# Autodesk Inventor assembly: left_leg_MIR
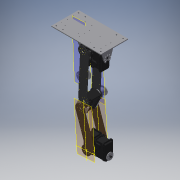
[picture p0: Inventor's stored thumbnail of the model, 180x180]
Saved by Autodesk Inventor 2018 (Build 220112000, 112)
## iProperties
Created: 2018-11-26
Part Number: left_leg_MIR
Document SubType Name: Assembly
Designer: bitbots
Mass: 578.906 g
Surface Area: 2185.74 cm^2
Volume: 578.906 cm^3
Density: 1 g/cm^3
Author: bitbots
## Documents named in this file (14)
- C:\Users\bitbots\Desktop\bitbots_hardware\wolfgang\assembly\legs\left_leg.iam
- C:\Users\bitbots\Desktop\bitbots_hardware\wolfgang\assembly\legs\lower_leg_MIR.ipt
- C:\Users\bitbots\Desktop\bitbots_hardware\wolfgang\assembly\legs\upper_leg_MIR.ipt
- C:\Users\bitbots\Desktop\bitbots_hardware\wolfgang\assembly\motors\MX106\MX-106_with_bearing_MIR.iam
- C:\Users\bitbots\Desktop\bitbots_hardware\wolfgang\assembly\legs\knee_connector_MIR.ipt
- C:\Users\bitbots\Desktop\bitbots_hardware\wolfgang\assembly\legs\motor_connector_MIR.ipt
- C:\Users\bitbots\Desktop\bitbots_hardware\wolfgang\assembly\motors\MX106\MX-106_with_horn_MIR.iam
- C:\Users\bitbots\Desktop\bitbots_hardware\wolfgang\assembly\legs\ankle_MIR.ipt
- C:\Users\bitbots\Desktop\bitbots_hardware\wolfgang\assembly\legs\foot_MIR.ipt
- C:\Users\bitbots\Documents\spring_holder.ipt
- C:\Users\bitbots\Documents\springerholder_top.ipt
- C:\Users\bitbots\Documents\spring_holder_lower.ipt
- C:\Users\bitbots\Documents\springholder_new.ipt
- C:\Users\bitbots\Documents\springholder_new_bottom.ipt
## Components (22 placed, 13 different names)
1. lower_leg_MIR:1 — Mate:41, Mate:40, Mate:39, Mate:58, Mate:57, Flush:1, Flush:2, Flush:3, Flush:4, Flush:5, Flush:6, Mate:71, Mate:72, Mate:73
2. upper_leg_MIR:1 — Mate:33, Mate:32, Mate:31, Mate:35, Mate:34
3. lower_leg_MIR:2 — Mate:81, Mate:61, Mate:80, Mate:64
4. upper_leg_MIR:2 — Mate:82, Mate:28, Mate:38, Mate:37, Mate:36, Mate:52
5. MX-106_with_bearing_MIR:1 [sub-assembly] — Mate:81, Mate:61, Mate:41, Mate:40, Mate:39, Mate:22, Mate:21, Mate:20, Mate:18, Mate:17, Mate:16
6. MX-106_with_bearing_MIR:2 [sub-assembly] — Mate:82, Mate:33, Mate:32, Mate:31, Mate:29, Mate:28, Mate:10, Mate:9, Mate:8, Mate:7, Mate:6, Mate:5
7. knee_connector_MIR:1 — Mate:38, Mate:37, Mate:36, Mate:22, Mate:21, Mate:20, Mate:52
8. knee_connector_MIR:2 — Mate:35, Mate:34, Mate:18, Mate:17, Mate:16
9. motor_connector_MIR:1 — Mate:54, Mate:55, Mate:56, Mate:59, Mate:60, Mate:64
10. motor_connector_MIR:2 — Mate:73, Mate:57, Mate:58, Mate:61, Mate:62, Mate:63
11. motor_connector_MIR:3 — Mate:10, Mate:9, Mate:8, Mate:12, Mate:11
12. motor_connector_MIR:4 — Mate:7, Mate:6, Mate:5, Mate:13
13. MX-106_with_horn_MIR:1 [sub-assembly] — Mate:30, Mate:13, Mate:12, Mate:11, Angle:2
14. MX-106_with_bearing_MIR:3 [sub-assembly] — Mate:80, Mate:64, Mate:58, Mate:57, Mate:59, Mate:60, Mate:64
15. MX-106_with_horn_MIR:2 [sub-assembly] — Mate:73, Mate:54, Mate:55, Mate:56, Mate:57, Mate:58, Mate:61, Mate:62, Mate:63, Mate:65, Mate:66, Mate:67, Angle:2
16. ankle_MIR:1 — Mate:79, Mate:78, Mate:77, Mate:65, Mate:66, Mate:67
17. foot_MIR:1 — Mate:79, Mate:78, Mate:77, Angle:1
18. spring_holder:1 — Flush:1, Flush:2, Mate:68, Mate:69, Mate:70
19. springerholder_top:1 — Mate:68, Mate:69, Mate:70
20. spring_holder_lower:1 — Flush:3, Flush:4
21. springholder_new:1 — Flush:5, Flush:6, Mate:74, Mate:75, Mate:76
22. springholder_new_bottom:1 — Mate:71, Mate:72, Mate:73, Mate:74, Mate:75, Mate:76
## Relationships (72: Mate 64, Flush 6, Angle 2)
- Mate:81: lower_leg_MIR:2 ↔ MX-106_with_bearing_MIR:1
- Mate:61: lower_leg_MIR:2 ↔ MX-106_with_bearing_MIR:1
- Mate:41: lower_leg_MIR:1 ↔ MX-106_with_bearing_MIR:1
- Mate:40: lower_leg_MIR:1 ↔ MX-106_with_bearing_MIR:1
- Mate:39: lower_leg_MIR:1 ↔ MX-106_with_bearing_MIR:1
- Mate:82: upper_leg_MIR:2 ↔ MX-106_with_bearing_MIR:2
- Mate:33: upper_leg_MIR:1 ↔ MX-106_with_bearing_MIR:2
- Mate:32: upper_leg_MIR:1 ↔ MX-106_with_bearing_MIR:2
- Mate:31: upper_leg_MIR:1 ↔ MX-106_with_bearing_MIR:2
- Mate:29: MX-106_with_bearing_MIR:2
- Mate:28: upper_leg_MIR:2 ↔ MX-106_with_bearing_MIR:2
- Mate:38 (0.65 mm): upper_leg_MIR:2 ↔ knee_connector_MIR:1
- Mate:37: upper_leg_MIR:2 ↔ knee_connector_MIR:1
- Mate:36: upper_leg_MIR:2 ↔ knee_connector_MIR:1
- Mate:22: MX-106_with_bearing_MIR:1 ↔ knee_connector_MIR:1
- Mate:21: MX-106_with_bearing_MIR:1 ↔ knee_connector_MIR:1
- Mate:20: MX-106_with_bearing_MIR:1 ↔ knee_connector_MIR:1
- Mate:35: upper_leg_MIR:1 ↔ knee_connector_MIR:2
- Mate:34: upper_leg_MIR:1 ↔ knee_connector_MIR:2
- Mate:18: MX-106_with_bearing_MIR:1 ↔ knee_connector_MIR:2
- Mate:17: MX-106_with_bearing_MIR:1 ↔ knee_connector_MIR:2
- Mate:16: MX-106_with_bearing_MIR:1 ↔ knee_connector_MIR:2
- Mate:10: MX-106_with_bearing_MIR:2 ↔ motor_connector_MIR:3
- Mate:9: MX-106_with_bearing_MIR:2 ↔ motor_connector_MIR:3
- Mate:8: MX-106_with_bearing_MIR:2 ↔ motor_connector_MIR:3
- Mate:7: MX-106_with_bearing_MIR:2 ↔ motor_connector_MIR:4
- Mate:6: MX-106_with_bearing_MIR:2 ↔ motor_connector_MIR:4
- Mate:5: MX-106_with_bearing_MIR:2 ↔ motor_connector_MIR:4
- Mate:30: MX-106_with_horn_MIR:1
- Mate:13: motor_connector_MIR:4 ↔ MX-106_with_horn_MIR:1
- Mate:12: motor_connector_MIR:3 ↔ MX-106_with_horn_MIR:1
- Mate:11: motor_connector_MIR:3 ↔ MX-106_with_horn_MIR:1
- Mate:80: lower_leg_MIR:2 ↔ MX-106_with_bearing_MIR:3
- Mate:64: lower_leg_MIR:2 ↔ MX-106_with_bearing_MIR:3
- Mate:58: lower_leg_MIR:1 ↔ MX-106_with_bearing_MIR:3
- Mate:57: lower_leg_MIR:1 ↔ MX-106_with_bearing_MIR:3
- Mate:73: motor_connector_MIR:2 ↔ MX-106_with_horn_MIR:2
- Mate:79: ankle_MIR:1 ↔ foot_MIR:1
- Mate:78: ankle_MIR:1 ↔ foot_MIR:1
- Mate:77: ankle_MIR:1 ↔ foot_MIR:1
- Mate:52 (0.65 mm): upper_leg_MIR:2 ↔ knee_connector_MIR:1
- Mate:54: motor_connector_MIR:1 ↔ MX-106_with_horn_MIR:2
- Mate:55: motor_connector_MIR:1 ↔ MX-106_with_horn_MIR:2
- Mate:56: motor_connector_MIR:1 ↔ MX-106_with_horn_MIR:2
- Mate:57: motor_connector_MIR:2 ↔ MX-106_with_horn_MIR:2
- Mate:58: motor_connector_MIR:2 ↔ MX-106_with_horn_MIR:2
- Mate:59: motor_connector_MIR:1 ↔ MX-106_with_bearing_MIR:3
- Mate:60: motor_connector_MIR:1 ↔ MX-106_with_bearing_MIR:3
- Mate:61: motor_connector_MIR:2 ↔ MX-106_with_horn_MIR:2
- Mate:62: motor_connector_MIR:2 ↔ MX-106_with_horn_MIR:2
- Mate:63: motor_connector_MIR:2 ↔ MX-106_with_horn_MIR:2
- Mate:64: motor_connector_MIR:1 ↔ MX-106_with_bearing_MIR:3
- Angle:1 (0 deg): foot_MIR:1
- Mate:65: MX-106_with_horn_MIR:2 ↔ ankle_MIR:1
- Mate:66: MX-106_with_horn_MIR:2 ↔ ankle_MIR:1
- Mate:67: MX-106_with_horn_MIR:2 ↔ ankle_MIR:1
- Flush:1: lower_leg_MIR:1 ↔ spring_holder:1
- Flush:2: lower_leg_MIR:1 ↔ spring_holder:1
- Mate:68: spring_holder:1 ↔ springerholder_top:1
- Mate:69: spring_holder:1 ↔ springerholder_top:1
- Mate:70: spring_holder:1 ↔ springerholder_top:1
- Flush:3: lower_leg_MIR:1 ↔ spring_holder_lower:1
- Flush:4: lower_leg_MIR:1 ↔ spring_holder_lower:1
- Angle:2 (0 deg): MX-106_with_horn_MIR:1 ↔ MX-106_with_horn_MIR:2
- Flush:5: lower_leg_MIR:1 ↔ springholder_new:1
- Flush:6: lower_leg_MIR:1 ↔ springholder_new:1
- Mate:71: lower_leg_MIR:1 ↔ springholder_new_bottom:1
- Mate:72: lower_leg_MIR:1 ↔ springholder_new_bottom:1
- Mate:73: lower_leg_MIR:1 ↔ springholder_new_bottom:1
- Mate:74: springholder_new:1 ↔ springholder_new_bottom:1
- Mate:75: springholder_new:1 ↔ springholder_new_bottom:1
- Mate:76: springholder_new:1 ↔ springholder_new_bottom:1
